# Autodesk Inventor assembly: arm_assy_v3
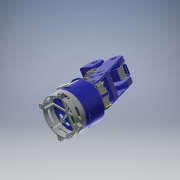
[picture p0: Inventor's stored thumbnail of the model, 180x180]
Saved by Autodesk Inventor 2018 (Build 220112000, 112)
## iProperties
Created: 2018-05-04
Part Number: arm_assy_v3
Document SubType Name: Assembly
Designer: mshaw2
Author: mshaw2
## Documents named in this file (26)
- C:\Users\mshaw2\OneDrive - University of Plymouth\ROCO224\arm_assy_v3.iam
- C:\Users\mshaw2\OneDrive - University of Plymouth\ROCO224\arm_segment_1_1c.ipt
- C:\Users\mshaw2\OneDrive - University of Plymouth\ROCO224\arm_segment_1_1d.ipt
- C:\Users\mshaw2\OneDrive - University of Plymouth\ROCO224\arm_segment_1_2c.ipt
- C:\Users\mshaw2\OneDrive - University of Plymouth\ROCO224\arm_segment_2_1.ipt
- C:\Users\mshaw2\OneDrive - University of Plymouth\ROCO224\arm_segment_3_2a.ipt
- C:\Users\mshaw2\OneDrive - University of Plymouth\ROCO224\arm_segment_3_2b.ipt
- C:\Users\mshaw2\OneDrive - University of Plymouth\ROCO224\base_enclosure_2.ipt
- C:\Users\mshaw2\OneDrive - University of Plymouth\ROCO224\base_turret_v3.ipt
- C:\Users\mshaw2\OneDrive - University of Plymouth\ROCO224\dual_motor_spacer_1.ipt
- C:\Users\mshaw2\OneDrive - University of Plymouth\ROCO224\grabber_rotating_mount_1.ipt
- C:\Users\mshaw2\OneDrive - University of Plymouth\ROCO224\RPI3B+.ipt
- C:\Users\mshaw2\OneDrive - University of Plymouth\ROCO224\ENS_SERVO-RX-28.iam
- C:\Users\mshaw2\OneDrive - University of Plymouth\ROCO224\base_1.ipt
- C:\Users\mshaw2\OneDrive - University of Plymouth\ROCO224\base_enclosure_1.ipt
- C:\Users\mshaw2\OneDrive - University of Plymouth\ROCO224\Component1.ipt
- C:\Users\mshaw2\OneDrive - University of Plymouth\ROCO224\Component2.ipt
- C:\Users\mshaw2\OneDrive - University of Plymouth\ROCO224\Component3.ipt
- C:\Users\mshaw2\Documents\Inventor\Content Center Files\R2018\en-US\SS-ISO 4762\ISO 4762 - M2.5 x 4SS-ISO.ipt
- C:\Users\mshaw2\Documents\Inventor\Content Center Files\R2018\en-US\SS-ISO 4762\ISO 4762 - M2.5 x 8SS-ISO.ipt
- C:\Users\mshaw2\Documents\Inventor\Content Center Files\R2018\en-US\SS-ISO 4762\ISO 4762 - M2 x 6SS-ISO.ipt
- C:\Users\mshaw2\Documents\Inventor\Content Center Files\R2018\en-US\SS-ISO 4762\ISO 4762 - M6 x 60SS-ISO.ipt
- C:\Users\mshaw2\Documents\Inventor\Content Center Files\R2018\en-US\SS-ISO 4762\ISO 4762 - M6 x 25SS-ISO.ipt
- C:\Users\mshaw2\Documents\Inventor\Content Center Files\R2018\en-US\SS-ISO 4762\ISO 4762 - M2.5 x 6SS-ISO.ipt
- C:\Users\mshaw2\Documents\Inventor\Content Center Files\R2018\en-US\ISO 4032(2)\ISO 4032 - M6 - ISO.ipt
- C:\Users\mshaw2\OneDrive - University of Plymouth\ROCO224\arm_gopro_mount_1.ipt
## Components (113 placed, 25 different names)
1. arm_segment_1_1c:1 — Rotational:2, Rigid:8, Angle:2, Insert:49, Insert:50, Insert:51, Insert:52, Insert:53, Insert:54, Insert:55, Insert:56, Insert:83, Insert:84, Insert:85
2. arm_segment_1_1d:1 — Rigid:8, Rigid:9, Insert:57, Insert:58, Insert:59, Insert:60, Insert:61, Insert:62, Insert:63, Insert:64, Insert:65, Insert:66, Insert:86
3. arm_segment_1_2c:1 — Rigid:10, Angle:1, Insert:81
4. arm_segment_2_1:1 — Rigid:12, Insert:17, Insert:18, Insert:19, Insert:20, Insert:21, Insert:22, Insert:23, Insert:24, Insert:25, Insert:26, Insert:27, Insert:28, Insert:29, Insert:30, Insert:31, Insert:32
5. arm_segment_1_2c:2 — Rigid:9, Rotational:3, Rigid:10, Insert:82
6. arm_segment_2_1:2 — Rigid:11, Rigid:14, Angle:1, Angle:3, Insert:33, Insert:34, Insert:35, Insert:36, Insert:37, Insert:38, Insert:39, Insert:40, Insert:41, Insert:42, Insert:43, Insert:44, Insert:45, Insert:46, Insert:47, Insert:48
7. arm_segment_3_2a:1 — Rotational:5, Rigid:13, Rigid:15, Insert:9, Insert:10, Insert:11, Insert:12, Insert:13, Insert:14, Insert:15, Insert:16
8. arm_segment_3_2b:1 — Rigid:13, Angle:3, Insert:1, Insert:2, Insert:3, Insert:4, Insert:5, Insert:6, Insert:7, Insert:8
9. base_enclosure_2:1 — Rigid:1, Rigid:2, Rigid:3
10. base_turret_v3:1 — Rotational:1, Rigid:5, Angle:2, Insert:67, Insert:68, Insert:69, Insert:70
11. dual_motor_spacer_1:1 — Rigid:6, Rigid:7
12. grabber_rotating_mount_1:1 — Rotational:6, Rigid:16
13. RPI3B+:1 — Rigid:2
14. base_1:1 — Mate:1, Mate:2, Rigid:1
15. base_enclosure_1:1 — Rigid:3, Rigid:4
16. Component1:1 — Rotational:7
17. Component2:1 — Rigid:17, Slider:1, Slider:2, Flush:1, Flush:2
18. Component3:1 — Slider:1, Flush:2
19. Component3:2 — Slider:2, Flush:1
20. SS ISO 4762 M2 x 6:1 — Insert:1
21. SS ISO 4762 M2 x 6:2 — Insert:2
22. SS ISO 4762 M2 x 6:3 — Insert:3
23. SS ISO 4762 M2 x 6:4 — Insert:4
24. SS ISO 4762 M2 x 6:5 — Insert:5
25. SS ISO 4762 M2 x 6:6 — Insert:6
26. SS ISO 4762 M2 x 6:7 — Insert:7
27. SS ISO 4762 M2 x 6:8 — Insert:8
28. SS ISO 4762 M2 x 6:9 — Insert:9
29. SS ISO 4762 M2 x 6:10 — Insert:10
30. SS ISO 4762 M2 x 6:11 — Insert:11
31. SS ISO 4762 M2 x 6:12 — Insert:12
32. SS ISO 4762 M2 x 6:13 — Insert:13
33. SS ISO 4762 M2 x 6:14 — Insert:14
34. SS ISO 4762 M2 x 6:15 — Insert:15
35. SS ISO 4762 M2 x 6:16 — Insert:16
36. SS ISO 4762 M2.5 x 8:1 — Insert:17
37. SS ISO 4762 M2.5 x 8:2 — Insert:18
38. SS ISO 4762 M2.5 x 8:3 — Insert:19
39. SS ISO 4762 M2.5 x 8:4 — Insert:20
40. SS ISO 4762 M2.5 x 8:5 — Insert:21
41. SS ISO 4762 M2.5 x 8:6 — Insert:22
42. SS ISO 4762 M2.5 x 8:7 — Insert:23
43. SS ISO 4762 M2.5 x 8:8 — Insert:24
44. SS ISO 4762 M2.5 x 8:9 — Insert:25
45. SS ISO 4762 M2.5 x 8:10 — Insert:26
46. SS ISO 4762 M2.5 x 8:11 — Insert:27
47. SS ISO 4762 M2.5 x 8:12 — Insert:28
48. SS ISO 4762 M2.5 x 8:13 — Insert:29
49. SS ISO 4762 M2.5 x 8:14 — Insert:30
50. SS ISO 4762 M2.5 x 8:15 — Insert:31
51. SS ISO 4762 M2.5 x 8:16 — Insert:32
52. SS ISO 4762 M2.5 x 8:17 — Insert:33
53. SS ISO 4762 M2.5 x 8:18 — Insert:34
54. SS ISO 4762 M2.5 x 8:19 — Insert:35
55. SS ISO 4762 M2.5 x 8:20 — Insert:36
56. SS ISO 4762 M2.5 x 8:21 — Insert:37
57. SS ISO 4762 M2.5 x 8:22 — Insert:38
58. SS ISO 4762 M2.5 x 8:23 — Insert:39
59. SS ISO 4762 M2.5 x 8:24 — Insert:40
60. SS ISO 4762 M2.5 x 8:25 — Insert:41
61. SS ISO 4762 M2.5 x 8:26 — Insert:42
62. SS ISO 4762 M2.5 x 8:27 — Insert:43
63. SS ISO 4762 M2.5 x 8:28 — Insert:44
64. SS ISO 4762 M2.5 x 8:29 — Insert:45
65. SS ISO 4762 M2.5 x 8:30 — Insert:46
66. SS ISO 4762 M2.5 x 8:31 — Insert:47
67. SS ISO 4762 M2.5 x 8:32 — Insert:48
68. SS ISO 4762 M2 x 6:17 — Insert:49
69. SS ISO 4762 M2 x 6:18 — Insert:50
70. SS ISO 4762 M2 x 6:19 — Insert:51
71. SS ISO 4762 M2 x 6:20 — Insert:52
72. SS ISO 4762 M2 x 6:21 — Insert:53
73. SS ISO 4762 M2 x 6:22 — Insert:54
74. SS ISO 4762 M2 x 6:23 — Insert:55
75. SS ISO 4762 M2 x 6:24 — Insert:56
76. SS ISO 4762 M2 x 6:25 — Insert:57
77. SS ISO 4762 M2 x 6:26 — Insert:58
78. SS ISO 4762 M2 x 6:27 — Insert:59
79. SS ISO 4762 M2 x 6:28 — Insert:60
80. SS ISO 4762 M2 x 6:29 — Insert:61
81. SS ISO 4762 M2 x 6:30 — Insert:62
82. SS ISO 4762 M2 x 6:31 — Insert:63
83. SS ISO 4762 M2 x 6:32 — Insert:64
84. SS ISO 4762 M6 x 60:1 — Insert:65
85. SS ISO 4762 M6 x 60:2 — Insert:66
86. SS ISO 4762 M2.5 x 4:1 — Insert:67
87. SS ISO 4762 M2.5 x 4:2 — Insert:68
88. SS ISO 4762 M2.5 x 4:3 — Insert:69
89. SS ISO 4762 M2.5 x 4:4 — Insert:70
90. SS ISO 4762 M2.5 x 6:1 — Insert:71
91. SS ISO 4762 M2.5 x 6:2 — Insert:72
92. SS ISO 4762 M2.5 x 6:3 — Insert:73
93. SS ISO 4762 M2.5 x 6:4 — Insert:74
94. SS ISO 4762 M2.5 x 6:5 — Insert:75
95. SS ISO 4762 M2.5 x 6:6 — Insert:76
96. SS ISO 4762 M2.5 x 6:7 — Insert:77
97. SS ISO 4762 M2.5 x 6:8 — Insert:78
98. SS ISO 4762 M2.5 x 6:9 — Insert:79
99. SS ISO 4762 M2.5 x 6:10 — Insert:80
100. SS ISO 4762 M6 x 25:1 — Insert:81
101. SS ISO 4762 M6 x 25:2 — Insert:82
102. ISO 4032 M6:1 — Insert:83
103. ISO 4032 M6:2 — Insert:84
104. ISO 4032 M6:3 — Insert:85
105. ISO 4032 M6:4 — Insert:86
106. arm_gopro_mount_1:1 — Rigid:18
107. ENS_SERVO-RX-28:7 [sub-assembly] — Rigid:16, Rigid:17, Rotational:7
108. ENS_SERVO-RX-28:1 [sub-assembly] — Rigid:4, Rotational:1
109. ENS_SERVO-RX-28:2 [sub-assembly] — Rigid:5, Rigid:6, Rotational:2, Insert:72, Insert:77, Insert:78, Insert:79, Insert:80
110. ENS_SERVO-RX-28:3 [sub-assembly] — Rigid:7, Insert:71, Insert:73, Insert:74, Insert:75, Insert:76
111. ENS_SERVO-RX-28:4 [sub-assembly] — Rotational:3, Rigid:11
112. ENS_SERVO-RX-28:5 [sub-assembly] — Rigid:14, Rigid:12, Rotational:5
113. ENS_SERVO-RX-28:6 [sub-assembly] — Rigid:15, Rotational:6, Rigid:18
## Relationships (119: Insert 86, WeldJoint 18, RevoluteJoint 6, Angle 3, Mate 2, TranslationJoint 2, Flush 2)
- Mate:1: base_1:1
- Mate:2: base_1:1
- Rigid:1 [WeldJoint]: base_enclosure_2:1 ↔ base_1:1
- Rigid:2 [WeldJoint]: base_enclosure_2:1 ↔ RPI3B+:1
- Rigid:3 [WeldJoint]: base_enclosure_2:1 ↔ base_enclosure_1:1
- Rigid:4 [WeldJoint]: base_enclosure_1:1 ↔ ENS_SERVO-RX-28:1
- Rotational:1 [RevoluteJoint]: base_turret_v3:1 ↔ ENS_SERVO-RX-28:1
- Rigid:5 [WeldJoint]: base_turret_v3:1 ↔ ENS_SERVO-RX-28:2
- Rigid:6 [WeldJoint]: dual_motor_spacer_1:1 ↔ ENS_SERVO-RX-28:2
- Rigid:7 [WeldJoint]: dual_motor_spacer_1:1 ↔ ENS_SERVO-RX-28:3
- Rotational:2 [RevoluteJoint]: arm_segment_1_1c:1 ↔ ENS_SERVO-RX-28:2
- Rigid:8 [WeldJoint]: arm_segment_1_1c:1 ↔ arm_segment_1_1d:1
- Rigid:9 [WeldJoint] (0.3 mm): arm_segment_1_1d:1 ↔ arm_segment_1_2c:2
- Rotational:3 [RevoluteJoint]: arm_segment_1_2c:2 ↔ ENS_SERVO-RX-28:4
- Rigid:10 [WeldJoint]: arm_segment_1_2c:1 ↔ arm_segment_1_2c:2
- Rigid:11 [WeldJoint]: arm_segment_2_1:2 ↔ ENS_SERVO-RX-28:4
- Rigid:14 [WeldJoint]: arm_segment_2_1:2 ↔ ENS_SERVO-RX-28:5
- Rigid:12 [WeldJoint]: arm_segment_2_1:1 ↔ ENS_SERVO-RX-28:5
- Rotational:5 [RevoluteJoint]: arm_segment_3_2a:1 ↔ ENS_SERVO-RX-28:5
- Rigid:13 [WeldJoint]: arm_segment_3_2a:1 ↔ arm_segment_3_2b:1
- Rigid:15 [WeldJoint]: arm_segment_3_2a:1 ↔ ENS_SERVO-RX-28:6
- Rotational:6 [RevoluteJoint]: grabber_rotating_mount_1:1 ↔ ENS_SERVO-RX-28:6
- Rigid:16 [WeldJoint]: grabber_rotating_mount_1:1 ↔ ENS_SERVO-RX-28:7
- Rigid:17 [WeldJoint]: Component2:1 ↔ ENS_SERVO-RX-28:7
- Rotational:7 [RevoluteJoint]: Component1:1 ↔ ENS_SERVO-RX-28:7
- Slider:1 [TranslationJoint]: Component2:1 ↔ Component3:1
- Slider:2 [TranslationJoint]: Component2:1 ↔ Component3:2
- Flush:1: Component2:1 ↔ Component3:2
- Flush:2: Component2:1 ↔ Component3:1
- Angle:1 (60 deg): arm_segment_1_2c:1 ↔ arm_segment_2_1:2
- Angle:2 (-120 deg): arm_segment_1_1c:1 ↔ base_turret_v3:1
- Angle:3 (90 deg): arm_segment_2_1:2 ↔ arm_segment_3_2b:1
- Insert:1: arm_segment_3_2b:1 ↔ SS ISO 4762 M2 x 6:1
- Insert:2: arm_segment_3_2b:1 ↔ SS ISO 4762 M2 x 6:2
- Insert:3: arm_segment_3_2b:1 ↔ SS ISO 4762 M2 x 6:3
- Insert:4: arm_segment_3_2b:1 ↔ SS ISO 4762 M2 x 6:4
- Insert:5: arm_segment_3_2b:1 ↔ SS ISO 4762 M2 x 6:5
- Insert:6: arm_segment_3_2b:1 ↔ SS ISO 4762 M2 x 6:6
- Insert:7: arm_segment_3_2b:1 ↔ SS ISO 4762 M2 x 6:7
- Insert:8: arm_segment_3_2b:1 ↔ SS ISO 4762 M2 x 6:8
- Insert:9: arm_segment_3_2a:1 ↔ SS ISO 4762 M2 x 6:9
- Insert:10: arm_segment_3_2a:1 ↔ SS ISO 4762 M2 x 6:10
- Insert:11: arm_segment_3_2a:1 ↔ SS ISO 4762 M2 x 6:11
- Insert:12: arm_segment_3_2a:1 ↔ SS ISO 4762 M2 x 6:12
- Insert:13: arm_segment_3_2a:1 ↔ SS ISO 4762 M2 x 6:13
- Insert:14: arm_segment_3_2a:1 ↔ SS ISO 4762 M2 x 6:14
- Insert:15: arm_segment_3_2a:1 ↔ SS ISO 4762 M2 x 6:15
- Insert:16: arm_segment_3_2a:1 ↔ SS ISO 4762 M2 x 6:16
- Insert:17: arm_segment_2_1:1 ↔ SS ISO 4762 M2.5 x 8:1
- Insert:18: arm_segment_2_1:1 ↔ SS ISO 4762 M2.5 x 8:2
- Insert:19: arm_segment_2_1:1 ↔ SS ISO 4762 M2.5 x 8:3
- Insert:20: arm_segment_2_1:1 ↔ SS ISO 4762 M2.5 x 8:4
- Insert:21: arm_segment_2_1:1 ↔ SS ISO 4762 M2.5 x 8:5
- Insert:22: arm_segment_2_1:1 ↔ SS ISO 4762 M2.5 x 8:6
- Insert:23: arm_segment_2_1:1 ↔ SS ISO 4762 M2.5 x 8:7
- Insert:24: arm_segment_2_1:1 ↔ SS ISO 4762 M2.5 x 8:8
- Insert:25: arm_segment_2_1:1 ↔ SS ISO 4762 M2.5 x 8:9
- Insert:26: arm_segment_2_1:1 ↔ SS ISO 4762 M2.5 x 8:10
- Insert:27: arm_segment_2_1:1 ↔ SS ISO 4762 M2.5 x 8:11
- Insert:28: arm_segment_2_1:1 ↔ SS ISO 4762 M2.5 x 8:12
- Insert:29: arm_segment_2_1:1 ↔ SS ISO 4762 M2.5 x 8:13
- Insert:30: arm_segment_2_1:1 ↔ SS ISO 4762 M2.5 x 8:14
- Insert:31: arm_segment_2_1:1 ↔ SS ISO 4762 M2.5 x 8:15
- Insert:32: arm_segment_2_1:1 ↔ SS ISO 4762 M2.5 x 8:16
- Insert:33: arm_segment_2_1:2 ↔ SS ISO 4762 M2.5 x 8:17
- Insert:34: arm_segment_2_1:2 ↔ SS ISO 4762 M2.5 x 8:18
- Insert:35: arm_segment_2_1:2 ↔ SS ISO 4762 M2.5 x 8:19
- Insert:36: arm_segment_2_1:2 ↔ SS ISO 4762 M2.5 x 8:20
- Insert:37: arm_segment_2_1:2 ↔ SS ISO 4762 M2.5 x 8:21
- Insert:38: arm_segment_2_1:2 ↔ SS ISO 4762 M2.5 x 8:22
- Insert:39: arm_segment_2_1:2 ↔ SS ISO 4762 M2.5 x 8:23
- Insert:40: arm_segment_2_1:2 ↔ SS ISO 4762 M2.5 x 8:24
- Insert:41: arm_segment_2_1:2 ↔ SS ISO 4762 M2.5 x 8:25
- Insert:42: arm_segment_2_1:2 ↔ SS ISO 4762 M2.5 x 8:26
- Insert:43: arm_segment_2_1:2 ↔ SS ISO 4762 M2.5 x 8:27
- Insert:44: arm_segment_2_1:2 ↔ SS ISO 4762 M2.5 x 8:28
- Insert:45: arm_segment_2_1:2 ↔ SS ISO 4762 M2.5 x 8:29
- Insert:46: arm_segment_2_1:2 ↔ SS ISO 4762 M2.5 x 8:30
- Insert:47: arm_segment_2_1:2 ↔ SS ISO 4762 M2.5 x 8:31
- Insert:48: arm_segment_2_1:2 ↔ SS ISO 4762 M2.5 x 8:32
- Insert:49: arm_segment_1_1c:1 ↔ SS ISO 4762 M2 x 6:17
- Insert:50: arm_segment_1_1c:1 ↔ SS ISO 4762 M2 x 6:18
- Insert:51: arm_segment_1_1c:1 ↔ SS ISO 4762 M2 x 6:19
- Insert:52: arm_segment_1_1c:1 ↔ SS ISO 4762 M2 x 6:20
- Insert:53: arm_segment_1_1c:1 ↔ SS ISO 4762 M2 x 6:21
- Insert:54: arm_segment_1_1c:1 ↔ SS ISO 4762 M2 x 6:22
- Insert:55: arm_segment_1_1c:1 ↔ SS ISO 4762 M2 x 6:23
- Insert:56: arm_segment_1_1c:1 ↔ SS ISO 4762 M2 x 6:24
- Insert:57: arm_segment_1_1d:1 ↔ SS ISO 4762 M2 x 6:25
- Insert:58: arm_segment_1_1d:1 ↔ SS ISO 4762 M2 x 6:26
- Insert:59: arm_segment_1_1d:1 ↔ SS ISO 4762 M2 x 6:27
- Insert:60: arm_segment_1_1d:1 ↔ SS ISO 4762 M2 x 6:28
- Insert:61: arm_segment_1_1d:1 ↔ SS ISO 4762 M2 x 6:29
- Insert:62: arm_segment_1_1d:1 ↔ SS ISO 4762 M2 x 6:30
- Insert:63: arm_segment_1_1d:1 ↔ SS ISO 4762 M2 x 6:31
- Insert:64: arm_segment_1_1d:1 ↔ SS ISO 4762 M2 x 6:32
- Insert:65: arm_segment_1_1d:1 ↔ SS ISO 4762 M6 x 60:1
- Insert:66: arm_segment_1_1d:1 ↔ SS ISO 4762 M6 x 60:2
- Insert:67: base_turret_v3:1 ↔ SS ISO 4762 M2.5 x 4:1
- Insert:68: base_turret_v3:1 ↔ SS ISO 4762 M2.5 x 4:2
- Insert:69: base_turret_v3:1 ↔ SS ISO 4762 M2.5 x 4:3
- Insert:70: base_turret_v3:1 ↔ SS ISO 4762 M2.5 x 4:4
- Insert:71: SS ISO 4762 M2.5 x 6:1 ↔ ENS_SERVO-RX-28:3
- Insert:72: SS ISO 4762 M2.5 x 6:2 ↔ ENS_SERVO-RX-28:2
- Insert:73: SS ISO 4762 M2.5 x 6:3 ↔ ENS_SERVO-RX-28:3
- Insert:74: SS ISO 4762 M2.5 x 6:4 ↔ ENS_SERVO-RX-28:3
- Insert:75: SS ISO 4762 M2.5 x 6:5 ↔ ENS_SERVO-RX-28:3
- Insert:76: SS ISO 4762 M2.5 x 6:6 ↔ ENS_SERVO-RX-28:3
- Insert:77: SS ISO 4762 M2.5 x 6:7 ↔ ENS_SERVO-RX-28:2
- Insert:78: SS ISO 4762 M2.5 x 6:8 ↔ ENS_SERVO-RX-28:2
- Insert:79: SS ISO 4762 M2.5 x 6:9 ↔ ENS_SERVO-RX-28:2
- Insert:80: SS ISO 4762 M2.5 x 6:10 ↔ ENS_SERVO-RX-28:2
- Insert:81: arm_segment_1_2c:1 ↔ SS ISO 4762 M6 x 25:1
- Insert:82: arm_segment_1_2c:2 ↔ SS ISO 4762 M6 x 25:2
- Insert:83: arm_segment_1_1c:1 ↔ ISO 4032 M6:1
- Insert:84: arm_segment_1_1c:1 ↔ ISO 4032 M6:2
- Insert:85: arm_segment_1_1c:1 ↔ ISO 4032 M6:3
- Insert:86: arm_segment_1_1d:1 ↔ ISO 4032 M6:4
- Rigid:18 [WeldJoint]: arm_gopro_mount_1:1 ↔ ENS_SERVO-RX-28:6
